# Autodesk Inventor assembly: AssBasedonStep
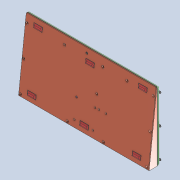
[picture p0: Inventor's stored thumbnail of the model, 180x180]
Saved by Autodesk Inventor 2022.3 (Build 263350030, 350C)
## iProperties
Created: 2022-11-01
Part Number: AssBasedonStep
Document SubType Name: Assembly
Designer: benka
Author: benka
## Documents named in this file (16)
- C:\GitHub\T420_KB_BLE\Enclosure\AssBasedonStep.iam
- C:\GitHub\T420_KB_BLE\Enclosure\BottomStep.ipt
- C:\GitHub\T420_KB_BLE\Enclosure\BezelStep2AfterFinal.ipt
- C:\GitHub\T420_KB_BLE\Enclosure\Elec.ipt
- C:\GitHub\T420_KB_BLE\Enclosure\5gram weight.ipt
- C:\GitHub\T420_KB_BLE\Enclosure\10gram weight.ipt
- C:\GitHub\T420_KB_BLE\Enclosure\Charger module_TC4056A_5V1A_USB Micro.ipt
- C:\GitHub\T420_KB_BLE\Enclosure\18650-battery-7.snapshot.1\18650 Battery Final.ipt
- C:\GitHub\T420_KB_BLE\Enclosure\m2 screw.ipt
- C:\GitHub\T420_KB_BLE\Enclosure\M3 Screw.ipt
- C:\GitHub\T420_KB_BLE\Enclosure\Pads.ipt
- C:\GitHub\T420_KB_BLE\Enclosure\Adafruit3258.ipt
- C:\Users\benka\University College London\AHRC - PBD Exhibitions - UCL_Code(Development) - UCL_Code(All)\0.Board Manufacturing&Box building\1.In-home manufacturing\Square Demo\pan_head_phillip_mc_screw_m2.ipt
- C:\GitHub\T420_KB_BLE\Enclosure\adafruit-bluefruit-le-uart-friend-bluetooth-low-energy-ble-1.snapshot.6\Adafruit_BlueFruit_UART_Rhino5\Adafruit_BlueFruit_UART2.ipt
- C:\GitHub\T420_KB_BLE\Enclosure\switch\Sliding Switch 2.ipt
- C:\GitHub\T420_KB_BLE\Enclosure\T420 Backplate Ben.ipt
## Components (32 placed, 15 different names)
1. BottomStep:1 — Mate:2, Mate:3, Flush:1, Rigid:2, Rigid:3, Mate:5, Mate:6, Mate:7, Mate:8, Mate:9, Mate:10, Mate:11, Mate:12, Mate:13, Mate:14, Mate:15, Mate:16, Mate:17, Mate:18, Mate:19, Mate:20, Mate:21, Mate:22, Mate:23, Mate:24, Mate:25, Mate:26, Rigid:4, Rigid:5, Rigid:6, Rigid:7, Rigid:8, Rigid:9, Mate:27, Mate:28, Mate:29, Cylindrical:1, Mate:30, Mate:31, Mate:32, Mate:33, Mate:34, Flush:2, Flush:3, Mate:36, Tangent:1, Flush:4
2. BezelStep2AfterFinal:1 — Mate:2, Mate:3, Angle:1
3. Elec:1 — Mate:28, Angle:1
4. 5gram weight:1 — Mate:33
5. 10gram weight:1 — Mate:32
6. Charger module_TC4056A_5V1A_USB Micro:1 — Mate:31
7. m2 screw:2 — Rigid:3, Mate:35
8. m2 screw:1 — Rigid:2
9. M3 Screw:1 — Mate:15, Mate:19
10. M3 Screw:2 — Mate:14, Mate:16
11. M3 Screw:3 — Mate:13, Mate:17
12. M3 Screw:4 — Mate:12, Mate:18
13. M3 Screw:5 — Mate:11, Mate:22
14. M3 Screw:6 — Mate:10, Mate:23
15. M3 Screw:7 — Mate:9, Mate:24
16. M3 Screw:8 — Mate:8, Mate:25
17. M3 Screw:9 — Mate:7, Mate:21
18. M3 Screw:10 — Mate:6, Mate:20
19. M3 Screw:11 — Mate:5, Mate:26
20. Pads:1 — Rigid:6
21. Pads:2 — Rigid:9
22. Pads:3 — Rigid:8
23. Pads:4 — Rigid:7
24. Pads:5 — Rigid:4
25. Pads:6 — Rigid:5
26. Adafruit3258:1 — Mate:27, Mate:29, Flush:3
27. pan_head_phillip_mc_screw_m2:1 — Cylindrical:1
28. Adafruit_BlueFruit_UART2:1 — Mate:30
29. Sliding Switch 2:1 — Mate:34, Flush:2
30. 18650 Battery Final:1 — Tangent:1, Flush:4
31. 18650 Battery Final:2
32. T420 Backplate Ben:1 — Mate:35, Mate:36
## Relationships (49: Mate 34, WeldJoint 8, Flush 4, Angle 1, CylindricalJoint 1, Tangent 1)
- Mate:2: BottomStep:1 ↔ BezelStep2AfterFinal:1
- Mate:3: BottomStep:1 ↔ BezelStep2AfterFinal:1
- Flush:1: BottomStep:1
- Rigid:2 [WeldJoint] (-0.79 mm): BottomStep:1 ↔ m2 screw:1
- Rigid:3 [WeldJoint] (-3.05 mm): BottomStep:1 ↔ m2 screw:2
- Mate:5: BottomStep:1 ↔ M3 Screw:11
- Mate:6: BottomStep:1 ↔ M3 Screw:10
- Mate:7: BottomStep:1 ↔ M3 Screw:9
- Mate:8: BottomStep:1 ↔ M3 Screw:8
- Mate:9: BottomStep:1 ↔ M3 Screw:7
- Mate:10: BottomStep:1 ↔ M3 Screw:6
- Mate:11: BottomStep:1 ↔ M3 Screw:5
- Mate:12: BottomStep:1 ↔ M3 Screw:4
- Mate:13: BottomStep:1 ↔ M3 Screw:3
- Mate:14: BottomStep:1 ↔ M3 Screw:2
- Mate:15: BottomStep:1 ↔ M3 Screw:1
- Mate:16: BottomStep:1 ↔ M3 Screw:2
- Mate:17: BottomStep:1 ↔ M3 Screw:3
- Mate:18: BottomStep:1 ↔ M3 Screw:4
- Mate:19: BottomStep:1 ↔ M3 Screw:1
- Mate:20: BottomStep:1 ↔ M3 Screw:10
- Mate:21: BottomStep:1 ↔ M3 Screw:9
- Mate:22: BottomStep:1 ↔ M3 Screw:5
- Mate:23: BottomStep:1 ↔ M3 Screw:6
- Mate:24: BottomStep:1 ↔ M3 Screw:7
- Mate:25: BottomStep:1 ↔ M3 Screw:8
- Mate:26: BottomStep:1 ↔ M3 Screw:11
- Rigid:4 [WeldJoint]: BottomStep:1 ↔ Pads:5
- Rigid:5 [WeldJoint]: BottomStep:1 ↔ Pads:6
- Rigid:6 [WeldJoint]: BottomStep:1 ↔ Pads:1
- Rigid:7 [WeldJoint]: BottomStep:1 ↔ Pads:4
- Rigid:8 [WeldJoint]: BottomStep:1 ↔ Pads:3
- Rigid:9 [WeldJoint]: BottomStep:1 ↔ Pads:2
- Mate:27 (-4 mm): BottomStep:1 ↔ Adafruit3258:1
- Mate:28 (3.5 mm): BottomStep:1 ↔ Elec:1
- Angle:1 (180 deg): BezelStep2AfterFinal:1 ↔ Elec:1
- Mate:29 (75 mm): BottomStep:1 ↔ Adafruit3258:1
- Cylindrical:1: BottomStep:1 ↔ pan_head_phillip_mc_screw_m2:1
- Mate:30 (3 mm): BottomStep:1 ↔ Adafruit_BlueFruit_UART2:1
- Mate:31: BottomStep:1 ↔ Charger module_TC4056A_5V1A_USB Micro:1
- Mate:32: BottomStep:1 ↔ 10gram weight:1
- Mate:33: BottomStep:1 ↔ 5gram weight:1
- Mate:34: BottomStep:1 ↔ Sliding Switch 2:1
- Flush:2 (-6.625 mm): BottomStep:1 ↔ Sliding Switch 2:1
- Flush:3 (4.5 mm): BottomStep:1 ↔ Adafruit3258:1
- Mate:35: m2 screw:2 ↔ T420 Backplate Ben:1
- Mate:36: BottomStep:1 ↔ T420 Backplate Ben:1
- Tangent:1: BottomStep:1 ↔ 18650 Battery Final:1
- Flush:4 (1 mm): BottomStep:1 ↔ 18650 Battery Final:1
